# Autodesk Inventor assembly: ASSY_REACTOR
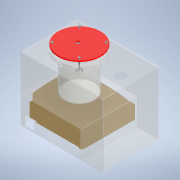
[picture p0: Inventor's stored thumbnail of the model, 180x180]
Saved by Autodesk Inventor 2021 (Build 250183000, 183)
## iProperties
Company: CHAROSA
Created: 2020-09-01
Part Number: ASSY_REACTOR
Document SubType Name: Assembly
Designer: C. SULLIVAN
Project: BIOLUMEN REACTOR
Checked By: C. SULLIVAN
Engr Approved By: C. SULLIVAN
Description: BIOLUMEN REACTOR, FULL ASSEMBLY WITH BEAKER CLAMP AND STIRRER; SENSORS OMITTED
Mfg Approved By: C. SULLIVAN
Engineer: C. SULLIVAN
Sending System: Creo  TM  6.0
Author: C. SULLIVAN
Title: ASSY, BIOLUMEN REACTOR
Revision Number: A
## Documents named in this file (4)
- C:\Users\Public\Documents\BioLumen Reactor\V2\Inventor_Versions\ASSY_REACTOR.iam
- C:\Users\Public\Documents\BioLumen Reactor\V2\Inventor_Versions\MAGNETIC_STIR_PLATE.ipt
- C:\Users\Public\Documents\BioLumen Reactor\V2\Inventor_Versions\ASSY_CLAMPING_RING.iam
- C:\Users\Public\Documents\BioLumen Reactor\V2\Inventor_Versions\ASSY_WATER_TANK.iam
## Components (3 placed, 3 different names)
1. ASSY_WATER_TANK [sub-assembly] — Insert:1
2. ASSY_CLAMPING_RING [sub-assembly] — Insert:1
3. MAGNETIC_STIR_PLATE
## Relationships (1: Insert 1)
- Insert:1: ASSY_WATER_TANK ↔ ASSY_CLAMPING_RING
